# Autodesk Inventor assembly: servo-mount
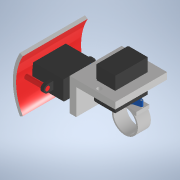
[picture p0: Inventor's stored thumbnail of the model, 180x180]
Saved by Autodesk Inventor 2022 (Build 260153000, 153)
## iProperties
Created: 2021-07-21
Part Number: servo-mount
Document SubType Name: Assembly
Designer: WASHINGTON
Author: WASHINGTON
## Documents named in this file (6)
- D:\TVC PAPER\servo-mount.iam
- D:\TVC PAPER\Servo\servo.ipt
- D:\TVC PAPER\Servo\servo horn.ipt
- D:\TVC PAPER\L-bracket.ipt
- D:\TVC PAPER\airframe - Copy.ipt
- D:\TVC PAPER\motor-hold.ipt
## Components (7 placed, 5 different names)
1. servo:1 — Mate:1, Mate:2, Mate:3, Mate:7, Mate:8, Mate:16, Mate:17
2. servo horn:1 — Mate:4, Mate:5, Mate:6, Mate:8, Mate:16, Mate:17
3. L-bracket:1 — Mate:4, Mate:5, Mate:6, Mate:7, Mate:10, Mate:12, Mate:18
4. airframe - Copy:1 — Mate:1, Mate:2, Mate:3
5. servo:2 — Mate:10, Mate:11, Mate:12, Mate:18
6. servo horn:2 — Mate:11, Mate:13, Mate:14, Mate:15
7. motor-hold:1 — Mate:13, Mate:14, Mate:15
## Relationships (18: Mate 18)
- Mate:1: servo:1 ↔ airframe - Copy:1
- Mate:2: servo:1 ↔ airframe - Copy:1
- Mate:3: servo:1 ↔ airframe - Copy:1
- Mate:4: servo horn:1 ↔ L-bracket:1
- Mate:5: servo horn:1 ↔ L-bracket:1
- Mate:6: servo horn:1 ↔ L-bracket:1
- Mate:7: servo:1 ↔ L-bracket:1
- Mate:8: servo:1 ↔ servo horn:1
- [Mate]: servo:2 ↔ servo horn:2
- Mate:10: L-bracket:1 ↔ servo:2
- Mate:11: servo:2 ↔ servo horn:2
- Mate:12: L-bracket:1 ↔ servo:2
- Mate:13: servo horn:2 ↔ motor-hold:1
- Mate:14: servo horn:2 ↔ motor-hold:1
- Mate:15: servo horn:2 ↔ motor-hold:1
- Mate:16: servo:1 ↔ servo horn:1
- Mate:17: servo:1 ↔ servo horn:1
- Mate:18: L-bracket:1 ↔ servo:2
## Named parameters: d11_d10 = 0 mm
